# Autodesk Inventor assembly: case
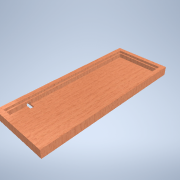
[picture p0: Inventor's stored thumbnail of the model, 180x180]
Saved by Autodesk Inventor 2022 (Build 260153000, 153)
## iProperties
Created: 2022-03-03
Part Number: case
Document SubType Name: Assembly
Designer: Nathan Griffith
Author: Nathan Griffith
## Documents named in this file (3)
- C:\Users\Nathan Griffith\Documents\Eric60percentkeyboard\Inventor\Case\case.iam
- C:\Users\Nathan Griffith\Documents\Eric60percentkeyboard\Inventor\Case stock 1.ipt
- C:\Users\Nathan Griffith\Documents\Eric60percentkeyboard\Inventor\Case\Case Parts.ipt
## Components (2 placed, 2 different names)
1. Case stock 1:1 — Flush:1, Flush:2
2. Case Parts:1 — Flush:1, Flush:2
## Relationships (2: Flush 2)
- Flush:1: Case stock 1:1 ↔ Case Parts:1
- Flush:2: Case stock 1:1 ↔ Case Parts:1
